# Autodesk Inventor assembly: pca_obudowa
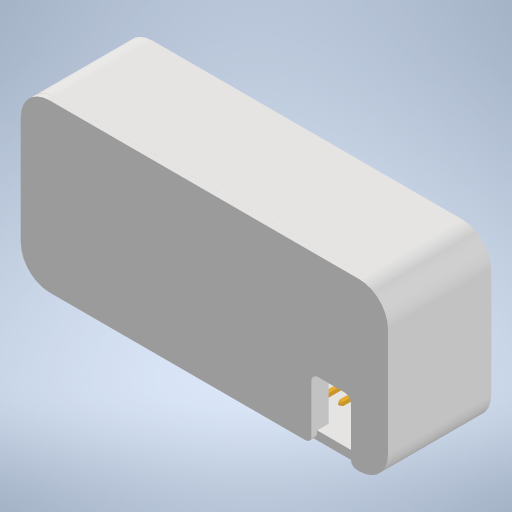
[picture p0: Inventor's stored thumbnail of the model, 512x512]
Saved by Autodesk Inventor 2023 (Build 270158000, 158)
## iProperties
Created: 2024-05-25
Part Number: pca_obudowa
Document SubType Name: Assembly
Designer: kamil
Author: kamil
## Documents named in this file (4)
- C:\Users\kamil\Documents\PROJECTS - repos\ModBot---Projekt-Zespolowy\mechanics\pca_obudowa.iam
- C:\Users\kamil\Documents\PROJECTS - repos\ModBot---Projekt-Zespolowy\mechanics\STEP\pca9685.ipt
- C:\Users\kamil\Documents\PROJECTS - repos\ModBot---Projekt-Zespolowy\mechanics\pca_obudowa_dol.ipt
- C:\Users\kamil\Documents\PROJECTS - repos\ModBot---Projekt-Zespolowy\mechanics\pca_obudowa_gora.ipt
## Components (3 placed, 3 different names)
1. pca9685:1 — Równoległe:1
2. pca_obudowa_dol:1 — Równoległe:1, Równoległe:2
3. pca_obudowa_gora:1 — Równoległe:2
## Relationships (2: Flush 2)
- Równoległe:1 [Flush]: pca9685:1 ↔ pca_obudowa_dol:1
- Równoległe:2 [Flush]: pca_obudowa_dol:1 ↔ pca_obudowa_gora:1
